# Autodesk Inventor assembly: extruder
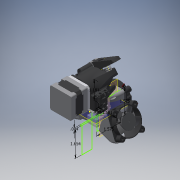
[picture p0: Inventor's stored thumbnail of the model, 180x180]
Saved by Autodesk Inventor 2017 (Build 210142000, 142)
## iProperties
Created: 2016-05-21
Part Number: extruder
Document SubType Name: Assembly
Designer: brent
Author: brent
## Documents named in this file (9)
- C:\Users\yibre\OneDrive\personal\printer_mechanical\extruder\extruder_175mm.iam
- C:\Users\yibre\OneDrive\personal\printer_mechanical\extruder\extruder_175mm.ipt
- C:\Users\yibre\OneDrive\personal\printer_mechanical\offtheshelf\gearedstepper.ipt
- C:\Users\yibre\OneDrive\personal\printer_mechanical\offtheshelf\mk8_drivegear.ipt
- C:\Users\yibre\OneDrive\personal\printer_mechanical\offtheshelf\extruder_spring.ipt
- C:\Users\yibre\OneDrive\personal\printer_mechanical\offtheshelf\623bearing.ipt
- C:\Users\yibre\OneDrive\personal\printer_mechanical\extruder\fan_shroud.ipt
- C:\Users\yibre\OneDrive\personal\printer_mechanical\offtheshelf\40mm_fan.ipt
- C:\Users\yibre\OneDrive\personal\printer_mechanical\extruder\hotend_alternative.ipt
## Components (12 placed, 8 different names)
1. extruder_175mm:1 — Mate:15, Flush:2, Mate:16, Mate:18, Mate:19, Mate:22, Mate:24, Mate:25, Mate:27, Mate:29, Flush:3, Mate:42, Mate:43, Angle:1
2. gearedstepper:1 — Mate:5, Mate:19, Mate:22, Mate:25, Mate:28
3. mk8_drivegear:1 — Mate:5, Mate:28
4. extruder_spring:1 — Mate:15, Flush:2
5. 623bearing:1 — Mate:18, Mate:29
6. 623bearing:2 — Mate:16, Mate:17, Mate:24
7. 623bearing:3 — Mate:17, Mate:27
8. fan_shroud:1 — Mate:33, Mate:34, Mate:35, Mate:36, Mate:37, Mate:38, Mate:39, Mate:40, Mate:41
9. 40mm_fan:1 — Mate:34, Mate:40, Mate:41
10. 40mm_fan:2 — Mate:35, Mate:36, Mate:37
11. 40mm_fan:3 — Mate:33, Mate:38, Mate:39
12. hotend_alternative:1 — Mate:42, Mate:43, Angle:1
## Relationships (26: Mate 23, Flush 2, Angle 1)
- Mate:5: gearedstepper:1 ↔ mk8_drivegear:1
- Mate:15: extruder_175mm:1 ↔ extruder_spring:1
- Flush:2: extruder_175mm:1 ↔ extruder_spring:1
- Mate:16: extruder_175mm:1 ↔ 623bearing:2
- Mate:17: 623bearing:2 ↔ 623bearing:3
- Mate:18: extruder_175mm:1 ↔ 623bearing:1
- Mate:19: extruder_175mm:1 ↔ gearedstepper:1
- Mate:22: extruder_175mm:1 ↔ gearedstepper:1
- Mate:24: extruder_175mm:1 ↔ 623bearing:2
- Mate:25: extruder_175mm:1 ↔ gearedstepper:1
- Mate:27: extruder_175mm:1 ↔ 623bearing:3
- Mate:28 (1.65 mm): gearedstepper:1 ↔ mk8_drivegear:1
- Mate:29 (0.3 mm): extruder_175mm:1 ↔ 623bearing:1
- Flush:3 (10 mm): extruder_175mm:1
- Mate:33: fan_shroud:1 ↔ 40mm_fan:3
- Mate:34: fan_shroud:1 ↔ 40mm_fan:1
- Mate:35: fan_shroud:1 ↔ 40mm_fan:2
- Mate:36: fan_shroud:1 ↔ 40mm_fan:2
- Mate:37 (1.6256 mm): fan_shroud:1 ↔ 40mm_fan:2
- Mate:38: fan_shroud:1 ↔ 40mm_fan:3
- Mate:39: fan_shroud:1 ↔ 40mm_fan:3
- Mate:40: fan_shroud:1 ↔ 40mm_fan:1
- Mate:41: fan_shroud:1 ↔ 40mm_fan:1
- Mate:42: extruder_175mm:1 ↔ hotend_alternative:1
- Mate:43: extruder_175mm:1 ↔ hotend_alternative:1
- Angle:1 (0 deg): extruder_175mm:1 ↔ hotend_alternative:1
